# Autodesk Inventor assembly: Ball Shifter shifting shaft with gears
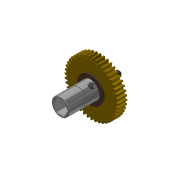
[picture p0: Inventor's stored thumbnail of the model, 180x180]
Saved by Autodesk Inventor 2013 (Build 170138000, 138)
## iProperties
Created: 2013-04-08
Part Number: Ball Shifter shifting shaft with gears
Document SubType Name: Assembly
Designer: Niemitalo_Dan
Author: Niemitalo_Dan
## Documents named in this file (4)
- H:\Nemo\Documents\Robotics\CAD Files\COTS Parts\Gearboxes\Components\Ballshifter\Ball Shifter shifting shaft with gears.iam
- H:\Nemo\Documents\Robotics\CAD Files\COTS Parts\Gearboxes\Components\Ballshifter\Ball Shifter Shaft assy.iam
- H:\Nemo\Documents\Robotics\CAD Files\COTS Parts\Gearboxes\Components\Ballshifter\Ballshifter shaft washer.ipt
- H:\Nemo\Documents\Robotics\CAD Files\COTS Parts\Gears - VexPro\Gear 20dp ball shifter 44T Vex.ipt
## Components (3 placed, 3 different names)
1. Ball Shifter Shaft assy:1 [sub-assembly] — Insert:1
2. Ballshifter shaft washer:1 — Insert:1, Insert:2
3. Gear 20dp ball shifter 44T Vex:1 — Insert:2
## Relationships (2: Insert 2)
- Insert:1: Ball Shifter Shaft assy:1 ↔ Ballshifter shaft washer:1
- Insert:2: Ballshifter shaft washer:1 ↔ Gear 20dp ball shifter 44T Vex:1
